# Autodesk Inventor assembly: Final_Assembly
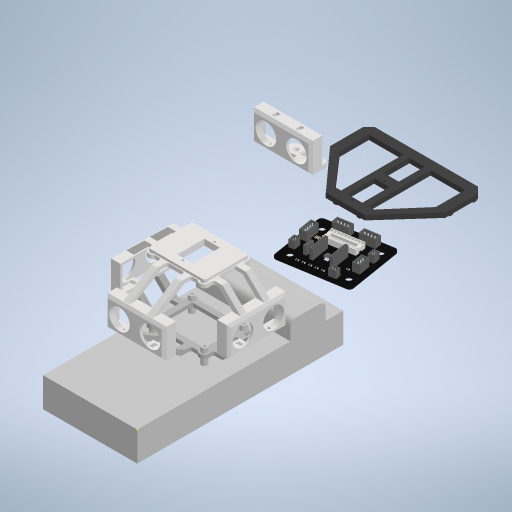
[picture p0: Inventor's stored thumbnail of the model, 512x512]
Saved by Autodesk Inventor 2024.2 (Build 282272000, 272)
## iProperties
Created: 2024-04-01
Part Number: Final_Assembly
Document SubType Name: Assembly
Designer: ringl
Author: ringl
## Documents named in this file (8)
- C:\Users\ringl\OneDrive\Uni_PC_backup\Y4S2\EE579\Assignment\EE579-Skittles\CAD\Final_Assembly.iam
- C:\Users\ringl\OneDrive\Uni_PC_backup\Y4S2\EE579\Assignment\EE579-Skittles\CAD\CarApproximation.ipt
- C:\Users\ringl\OneDrive\Uni_PC_backup\Y4S2\EE579\Assignment\EE579-Skittles\PCB\EE579_Skittles_pcb\EE579_Skittles_pcb.iam
- C:\Users\ringl\OneDrive\Uni_PC_backup\Y4S2\EE579\Assignment\EE579-Skittles\CAD\TopServoMount.ipt
- C:\Users\ringl\OneDrive\Uni_PC_backup\Y4S2\EE579\Assignment\EE579-Skittles\CAD\Full_Mount.ipt
- C:\Users\ringl\OneDrive\Uni_PC_backup\Y4S2\EE579\Assignment\EE579-Skittles\CAD\UltrasonicSensorMount.ipt
- C:\Users\ringl\OneDrive\Uni_PC_backup\Y4S2\EE579\Assignment\EE579-Skittles\CAD\ServoUltrasonicMount.ipt
- C:\Users\ringl\OneDrive\Uni_PC_backup\Y4S2\EE579\Assignment\EE579-Skittles\CAD\ServoFullMountInsert.ipt
## Components (12 placed, 7 different names)
1. CarApproximation:1 — Mate:1, Mate:2, Mate:3
2. EE579_Skittles_pcb:1 [sub-assembly] — Mate:1
3. TopServoMount:1
4. TopServoMount:2
5. Full_Mount:1 — Mate:2, Mate:3, Mate:4, Mate:5, Mate:6, Mate:7, Mate:8, Mate:9, Mate:10, Mate:11
6. UltrasonicSensorMount:1 — Mate:4, Mate:5, Mate:6
7. UltrasonicSensorMount:2 — Mate:7, Mate:8, Mate:9, Mate:16, Mate:17
8. UltrasonicSensorMount:3 — Mate:10, Mate:11, Mate:15
9. ServoUltrasonicMount:1 — Mate:12, Mate:13, Mate:14
10. UltrasonicSensorMount:4 — Mate:12, Mate:13, Mate:14
11. Full_Mount:2 — Mate:15, Mate:16, Mate:17, Mate:18, Mate:19
12. ServoFullMountInsert:1 — Mate:18, Mate:19
## Relationships (19: Mate 19)
- Mate:1 (10 mm): CarApproximation:1 ↔ EE579_Skittles_pcb:1
- Mate:2: CarApproximation:1 ↔ Full_Mount:1
- Mate:3: CarApproximation:1 ↔ Full_Mount:1
- Mate:4 (0.1 mm): Full_Mount:1 ↔ UltrasonicSensorMount:1
- Mate:5: Full_Mount:1 ↔ UltrasonicSensorMount:1
- Mate:6: Full_Mount:1 ↔ UltrasonicSensorMount:1
- Mate:7: Full_Mount:1 ↔ UltrasonicSensorMount:2
- Mate:8 (0.1 mm): Full_Mount:1 ↔ UltrasonicSensorMount:2
- Mate:9: Full_Mount:1 ↔ UltrasonicSensorMount:2
- Mate:10: Full_Mount:1 ↔ UltrasonicSensorMount:3
- Mate:11 (0.1 mm): Full_Mount:1 ↔ UltrasonicSensorMount:3
- Mate:12: ServoUltrasonicMount:1 ↔ UltrasonicSensorMount:4
- Mate:13: ServoUltrasonicMount:1 ↔ UltrasonicSensorMount:4
- Mate:14 (0.1 mm): ServoUltrasonicMount:1 ↔ UltrasonicSensorMount:4
- Mate:15: UltrasonicSensorMount:3 ↔ Full_Mount:2
- Mate:16: UltrasonicSensorMount:2 ↔ Full_Mount:2
- Mate:17 (0.1 mm): UltrasonicSensorMount:2 ↔ Full_Mount:2
- Mate:18: Full_Mount:2 ↔ ServoFullMountInsert:1
- Mate:19: Full_Mount:2 ↔ ServoFullMountInsert:1
